# Autodesk Inventor assembly: Wheel Assembly
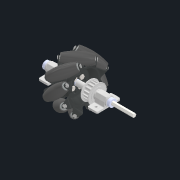
[picture p0: Inventor's stored thumbnail of the model, 180x180]
Saved by Autodesk Inventor 2022 (Build 260153000, 153)
## iProperties
Created: 2021-11-02
Part Number: Wheel Assembly
Document SubType Name: Assembly
Designer: divid
Author: divid
## Documents named in this file (12)
- C:\Users\divid\Documents\GitHub\ComputerAidedDesign\2021-22\FTC\#13822 Robovikes\Drivetrain\Wheel Assembly\Wheel Assembly (Right).iam
- C:\Users\divid\Documents\GitHub\ComputerAidedDesign\2021-22\FTC\#13822 Robovikes\Drivetrain\Wheel Assembly\15mm Bearing Pillow Block.ipt
- C:\Users\divid\Documents\GitHub\ComputerAidedDesign\2021-22\FTC\#13822 Robovikes\Drivetrain\Wheel Assembly\Through Bore Bearing - Short.ipt
- C:\Users\divid\Documents\GitHub\ComputerAidedDesign\2021-22\FTC\#13822 Robovikes\Drivetrain\Wheel Assembly\Through Bore Bearing - Long.ipt
- C:\Users\divid\Documents\GitHub\ComputerAidedDesign\2021-22\FTC\#13822 Robovikes\Duck Carousel\Slim Shaft Collar - 10 Pack.ipt
- C:\Users\divid\Documents\GitHub\ComputerAidedDesign\2021-22\FTC\#13822 Robovikes\Drivetrain\Wheel Assembly\Shaft Collars.ipt
- C:\Users\divid\Documents\GitHub\ComputerAidedDesign\2021-22\FTC\#13822 Robovikes\Drivetrain\Wheel Assembly\3mm Spacer.ipt
- C:\Users\divid\Documents\GitHub\ComputerAidedDesign\2021-22\FTC\#13822 Robovikes\Drivetrain\Wheel Assembly\15mm Spacer.ipt
- C:\Users\divid\Documents\GitHub\ComputerAidedDesign\2021-22\FTC\#13822 Robovikes\Drivetrain\Wheel Assembly\5mm x 135mm Hex Shaft.ipt
- C:\Users\divid\Documents\GitHub\ComputerAidedDesign\2021-22\FTC\#13822 Robovikes\Drivetrain\Wheel Assembly\Custom 5mm Hex Shaft Timing Belt Pulley\3414 Series Timing Belt Pulley (5mm Hex Bore, 16 Tooth).iam
- C:\Users\divid\Documents\GitHub\ComputerAidedDesign\2021-22\FTC\#13822 Robovikes\Drivetrain\Wheel Assembly\Slim Shaft Collar.ipt
- C:\Users\divid\Documents\GitHub\ComputerAidedDesign\2021-22\FTC\#13822 Robovikes\Drivetrain\75mm Mecanum Wheel - Right.ipt
## Components (16 placed, 11 different names)
1. 15mm Bearing Pillow Block:1 — Rotational:1, Mate:11, Flush:2
2. Through Bore Bearing - Long:1 — Rotational:1, Mate:7, Mate:8, Mate:9, Mate:12, Mate:15, Mate:52
3. Through Bore Bearing - Short:1 — Mate:9, Mate:10, Mate:11, Mate:14
4. Slim Shaft Collar - 10 Pack:1 — Mate:50, Mate:52
5. Shaft Collars:1 — Mate:12, Mate:14, Mate:17
6. 3mm Spacer:1 — Mate:20, Mate:21, Mate:22, Mate:23
7. 3mm Spacer:2 — Mate:15, Mate:16, Mate:17, Mate:21
8. 15mm Spacer:1 — Mate:30, Mate:31, Mate:32, Mate:35
9. 3mm Spacer:3 — Mate:33, Mate:34, Mate:35, Mate:38
10. 5mm x 135mm Hex Shaft:1 — Mate:1, Mate:2, Mate:8, Mate:10
11. 15mm Bearing Pillow Block:2 — Mate:42, Mate:43, Mate:46, Flush:2
12. Through Bore Bearing - Long:2 — Mate:44, Mate:45, Mate:46, Mate:49
13. Through Bore Bearing - Short:2 — Mate:39, Mate:40, Mate:41, Mate:43
14. Slim Shaft Collar:1 — Mate:47, Mate:49
15. 3414 Series Timing Belt Pulley (5mm Hex Bore, 16 Tooth):1 [sub-assembly] — Mate:36, Mate:37, Mate:38, Mate:41
16. 75mm Mecanum Wheel - Right:1 — Mate:18, Mate:19, Mate:23, Mate:32
## Relationships (42: Mate 40, RevoluteJoint 1, Flush 1)
- Rotational:1 [RevoluteJoint]: 15mm Bearing Pillow Block:1 ↔ Through Bore Bearing - Long:1
- Mate:1: 5mm x 135mm Hex Shaft:1
- Mate:2: 5mm x 135mm Hex Shaft:1
- Mate:5
- Mate:7: Through Bore Bearing - Long:1
- Mate:8: Through Bore Bearing - Long:1 ↔ 5mm x 135mm Hex Shaft:1
- Mate:9: Through Bore Bearing - Long:1 ↔ Through Bore Bearing - Short:1
- Mate:10: Through Bore Bearing - Short:1 ↔ 5mm x 135mm Hex Shaft:1
- Mate:11: 15mm Bearing Pillow Block:1 ↔ Through Bore Bearing - Short:1
- Mate:12: Through Bore Bearing - Long:1 ↔ Shaft Collars:1
- Mate:14: Through Bore Bearing - Short:1 ↔ Shaft Collars:1
- Mate:15: Through Bore Bearing - Long:1 ↔ 3mm Spacer:2
- Mate:16: 3mm Spacer:2
- Mate:17: Shaft Collars:1 ↔ 3mm Spacer:2
- Mate:18: 75mm Mecanum Wheel - Right:1
- Mate:19: 75mm Mecanum Wheel - Right:1
- Mate:20: 3mm Spacer:1
- Mate:21: 3mm Spacer:1 ↔ 3mm Spacer:2
- Mate:22: 3mm Spacer:1
- Mate:23: 3mm Spacer:1 ↔ 75mm Mecanum Wheel - Right:1
- Mate:30: 15mm Spacer:1
- Mate:31: 15mm Spacer:1
- Mate:32: 15mm Spacer:1 ↔ 75mm Mecanum Wheel - Right:1
- Mate:33: 3mm Spacer:3
- Mate:34: 3mm Spacer:3
- Mate:35: 15mm Spacer:1 ↔ 3mm Spacer:3
- Mate:36: 3414 Series Timing Belt Pulley (5mm Hex Bore, 16 Tooth):1
- Mate:37: 3414 Series Timing Belt Pulley (5mm Hex Bore, 16 Tooth):1
- Mate:38: 3mm Spacer:3 ↔ 3414 Series Timing Belt Pulley (5mm Hex Bore, 16 Tooth):1
- Mate:39: Through Bore Bearing - Short:2
- Mate:40: Through Bore Bearing - Short:2
- Mate:41: Through Bore Bearing - Short:2 ↔ 3414 Series Timing Belt Pulley (5mm Hex Bore, 16 Tooth):1
- Mate:42: 15mm Bearing Pillow Block:2
- Mate:43: 15mm Bearing Pillow Block:2 ↔ Through Bore Bearing - Short:2
- Mate:44: Through Bore Bearing - Long:2
- Mate:45: Through Bore Bearing - Long:2
- Mate:46: 15mm Bearing Pillow Block:2 ↔ Through Bore Bearing - Long:2
- Flush:2: 15mm Bearing Pillow Block:1 ↔ 15mm Bearing Pillow Block:2
- Mate:47: Slim Shaft Collar:1
- Mate:49: Through Bore Bearing - Long:2 ↔ Slim Shaft Collar:1
- Mate:50: Slim Shaft Collar - 10 Pack:1
- Mate:52: Through Bore Bearing - Long:1 ↔ Slim Shaft Collar - 10 Pack:1
